# Autodesk Inventor assembly: FP90-15deg
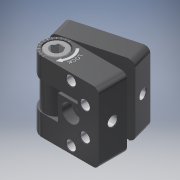
[picture p0: Inventor's stored thumbnail of the model, 180x180]
Saved by Autodesk Inventor 2019 (Build 230136000, 136)
## iProperties
Created: 2019-04-17
Part Number: FP90-15deg
Document SubType Name: Assembly
Designer: Wilson Lab
Author: Wilson Lab
## Documents named in this file (3)
- C:\code\auditory-behavior-experiments\design-files\vr-opto-assembly-2\FP90-15deg.iam
- C:\code\auditory-behavior-experiments\design-files\vr-opto-assembly\FP90-Solidworks-bottom.ipt
- C:\code\auditory-behavior-experiments\design-files\vr-opto-assembly\FP90-Solidworks-top.ipt
## Components (2 placed, 2 different names)
1. FP90-Solidworks-bottom:1 — Cylindrical:1, Mate:1
2. FP90-Solidworks-top:1 — Cylindrical:1, Mate:1
## Relationships (2: CylindricalJoint 1, Mate 1)
- Cylindrical:1: FP90-Solidworks-bottom:1 ↔ FP90-Solidworks-top:1
- Mate:1: FP90-Solidworks-bottom:1 ↔ FP90-Solidworks-top:1
